# Autodesk Inventor assembly: jetracer
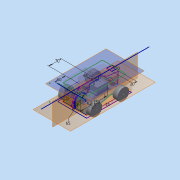
[picture p0: Inventor's stored thumbnail of the model, 180x180]
Saved by Autodesk Inventor 2022 (Build 260153000, 153)
## iProperties
Created: 2021-05-27
Part Number: jetracer
Material: Generisch
Document SubType Name: Assembly
Designer: Lukas
Author: Lukas
## Documents named in this file (11)
- E:\source\repos\S21\fachübergreifend\fennec bot\fennec-jet-racer\Konstruktion\jetracer.iam
- E:\source\repos\S21\fachübergreifend\fennec bot\fennec-jet-racer\Konstruktion\grundplatte.ipt
- E:\source\repos\S21\fachübergreifend\fennec bot\fennec-jet-racer\Konstruktion\waveshare_expansion_board.ipt
- E:\source\repos\S21\fachübergreifend\fennec bot\fennec-jet-racer\Konstruktion\abstandshalter_26mm.ipt
- E:\source\repos\S21\fachübergreifend\fennec bot\fennec-jet-racer\Konstruktion\abstandshalter_22mm.ipt
- E:\source\repos\S21\fachübergreifend\fennec bot\fennec-jet-racer\Konstruktion\jetson.ipt
- E:\source\repos\S21\fachübergreifend\fennec bot\fennec-jet-racer\Konstruktion\struktur.ipt
- E:\source\repos\S21\fachübergreifend\fennec bot\fennec-jet-racer\Konstruktion\reifen.ipt
- E:\source\repos\S21\fachübergreifend\fennec bot\fennec-jet-racer\Konstruktion\reifen_MIR.ipt
- E:\source\repos\S21\fachübergreifend\fennec bot\fennec-jet-racer\Konstruktion\chassis_front.ipt
- E:\source\repos\S21\fachübergreifend\fennec bot\fennec-jet-racer\Konstruktion\chassis_back.ipt
## Components (18 placed, 10 different names)
1. grundplatte:1 — Passend:1, Passend:2, Einfügen:1, Einfügen:2, Einfügen:3, Einfügen:4, Einfügen:5, Einfügen:6, Einfügen:7, Einfügen:8, Einfügen:9, Einfügen:10, Passend:3, Passend:4, Fluchtend:2, Fluchtend:3, Passend:6, Passend:7, Passend:11
2. waveshare_expansion_board:1 — Passend:2, Einfügen:1, Einfügen:2, Einfügen:11, Einfügen:12
3. abstandshalter_26mm:1 — Einfügen:6
4. abstandshalter_26mm:2 — Einfügen:3
5. abstandshalter_26mm:3 — Einfügen:5
6. abstandshalter_26mm:4 — Einfügen:4
7. abstandshalter_22mm:1 — Einfügen:10
8. abstandshalter_22mm:2 — Einfügen:9
9. abstandshalter_22mm:3 — Einfügen:7
10. abstandshalter_22mm:4 — Einfügen:8
11. jetson:1 — Einfügen:11, Einfügen:12, Fluchtend:4
12. struktur:1 — Fluchtend:2, Fluchtend:3, Fluchtend:4, Mate:10
13. reifen:1 — Passend:6, Passend:7
14. reifen_MIR:1
15. reifen:2
16. reifen_MIR:2
17. chassis_front:1 — Mate:10
18. chassis_back:1 — Passend:11, Passend:12
## Relationships (24: Insert 12, Mate 9, Flush 3)
- Passend:1 [Mate]: grundplatte:1
- Passend:2 [Mate] (26 mm): grundplatte:1 ↔ waveshare_expansion_board:1
- Einfügen:1 [Insert] (26 mm): grundplatte:1 ↔ waveshare_expansion_board:1
- Einfügen:2 [Insert] (26 mm): grundplatte:1 ↔ waveshare_expansion_board:1
- Einfügen:3 [Insert]: grundplatte:1 ↔ abstandshalter_26mm:2
- Einfügen:4 [Insert]: grundplatte:1 ↔ abstandshalter_26mm:4
- Einfügen:5 [Insert]: grundplatte:1 ↔ abstandshalter_26mm:3
- Einfügen:6 [Insert]: grundplatte:1 ↔ abstandshalter_26mm:1
- Einfügen:7 [Insert]: grundplatte:1 ↔ abstandshalter_22mm:3
- Einfügen:8 [Insert]: grundplatte:1 ↔ abstandshalter_22mm:4
- Einfügen:9 [Insert]: grundplatte:1 ↔ abstandshalter_22mm:2
- Einfügen:10 [Insert]: grundplatte:1 ↔ abstandshalter_22mm:1
- Einfügen:11 [Insert]: waveshare_expansion_board:1 ↔ jetson:1
- Passend:3 [Mate]: grundplatte:1
- Passend:4 [Mate]: grundplatte:1
- Einfügen:12 [Insert]: waveshare_expansion_board:1 ↔ jetson:1
- Fluchtend:2 [Flush]: grundplatte:1 ↔ struktur:1
- Fluchtend:3 [Flush]: grundplatte:1 ↔ struktur:1
- Fluchtend:4 [Flush]: jetson:1 ↔ struktur:1
- Passend:6 [Mate]: grundplatte:1 ↔ reifen:1
- Passend:7 [Mate] (5 mm): grundplatte:1 ↔ reifen:1
- Mate:10: struktur:1 ↔ chassis_front:1
- Passend:11 [Mate]: grundplatte:1 ↔ chassis_back:1
- Passend:12 [Mate]: chassis_back:1
